# Autodesk Inventor assembly: Move
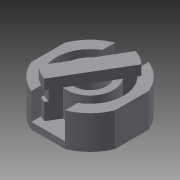
[picture p0: Inventor's stored thumbnail of the model, 180x180]
Saved by Autodesk Inventor 2015 (Build 190159000, 159)
## iProperties
Created: 2018-12-22
Part Number: Move
Document SubType Name: Assembly
Designer: kostya
Author: kostya
## Documents named in this file (3)
- C:\Users\kostya\source\repos\Models\Arkanoid\Ipt\Ather\Move.iam
- C:\Users\kostya\source\repos\Models\Arkanoid\Ipt\Ather\move female.ipt
- C:\Users\kostya\source\repos\Models\Arkanoid\Ipt\Ather\move male.ipt
## Components (2 placed, 2 different names)
1. move female:1 — Вставка:1
2. move male:1 — Вставка:1
## Relationships (1: Insert 1)
- Вставка:1 [Insert]: move female:1 ↔ move male:1
